# Autodesk Inventor assembly: EE_Assembly_Rev2
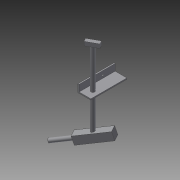
[picture p0: Inventor's stored thumbnail of the model, 180x180]
Saved by Autodesk Inventor 2015 (Build 190159000, 159)
## iProperties
Created: 2016-12-24
Part Number: EE_Assembly_Rev2
Document SubType Name: Assembly
Designer: Guy
Mass: 75.0572 g
Surface Area: 292.473 cm^2
Volume: 75.0572 cm^3
Density: 1 g/cm^3
Author: Guy
## Documents named in this file (4)
- C:\Users\Guy\Documents\Fourth Year\Capstone\git\Capstone-Project\doc\CAD\LowLevel_Rev2\EE_Assembly_Rev2.iam
- C:\Users\Guy\Documents\Fourth Year\Capstone\git\Capstone-Project\doc\CAD\LowLevel_Rev2\EE_Base-Rod-Rev2.ipt
- C:\Users\Guy\Documents\Fourth Year\Capstone\git\Capstone-Project\doc\CAD\LowLevel_Rev1\EE_Arm-Rod-Rev1.ipt
- C:\Users\Guy\Documents\Fourth Year\Capstone\git\Capstone-Project\doc\CAD\LowLevel_Rev1\EE-Rod-Rev1.ipt
## Components (3 placed, 3 different names)
1. EE_Base-Rod-Rev2:1 — Mate:1, Mate:2
2. EE_Arm-Rod-Rev1:1 — Mate:1, Mate:2, Mate:3, Flush:1, Mate:4, Mate:5
3. EE-Rod-Rev1:1 — Mate:3, Flush:1, Mate:4, Mate:5
## Relationships (6: Mate 5, Flush 1)
- Mate:1: EE_Base-Rod-Rev2:1 ↔ EE_Arm-Rod-Rev1:1
- Mate:2 (100 mm): EE_Base-Rod-Rev2:1 ↔ EE_Arm-Rod-Rev1:1
- Mate:3: EE_Arm-Rod-Rev1:1 ↔ EE-Rod-Rev1:1
- Flush:1 (5 mm): EE_Arm-Rod-Rev1:1 ↔ EE-Rod-Rev1:1
- Mate:4 (40 mm): EE_Arm-Rod-Rev1:1 ↔ EE-Rod-Rev1:1
- Mate:5 (40 mm): EE_Arm-Rod-Rev1:1 ↔ EE-Rod-Rev1:1
